# Autodesk Inventor assembly: Main_assembly
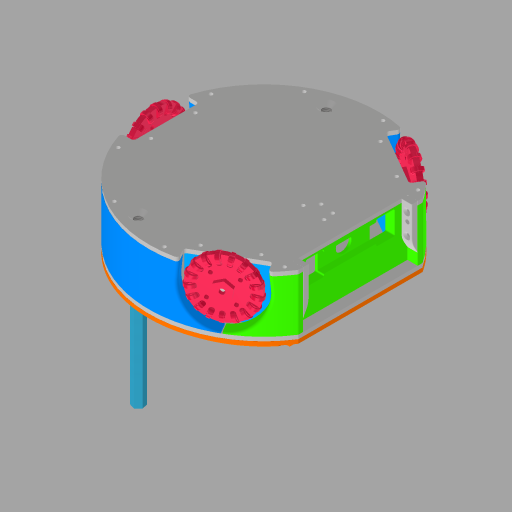
[picture p0: Inventor's stored thumbnail of the model, 512x512]
Saved by Autodesk Inventor 2024.2 (Build 282272000, 272)
## iProperties
Created: 2024-03-14
Part Number: Main_assembly
Document SubType Name: Assembly
Designer: Fedor Orlov
Author: Fedor Orlov
## Documents named in this file (18)
- C:\Users\Fedor Orlov\OneDrive\Robocup SSL\3D model\Main_assembly.iam
- C:\Users\Fedor Orlov\OneDrive\Robocup SSL\3D model\Level_1.ipt
- C:\Users\Fedor Orlov\OneDrive\Robocup SSL\3D model\Motor_mounting.ipt
- C:\Users\Fedor Orlov\OneDrive\Robocup SSL\3D model\Motor_mounting_left.ipt
- C:\Users\Fedor Orlov\OneDrive\Robocup SSL\3D model\Stand_M3_40mm.ipt
- C:\Users\Fedor Orlov\OneDrive\Robocup SSL\3D model\Stand_M6_40mm.ipt
- C:\Users\Fedor Orlov\OneDrive\Robocup SSL\3D model\Lower_protection_left.ipt
- C:\Users\Fedor Orlov\OneDrive\Robocup SSL\3D model\25d-metal-gearmotor-20.4.ipt
- C:\Users\Fedor Orlov\OneDrive\Robocup SSL\3D model\Lower_protection_right.ipt
- C:\Users\Fedor Orlov\OneDrive\Robocup SSL\3D model\gtf robots 50mm.ipt
- C:\Users\Fedor Orlov\OneDrive\Robocup SSL\3D model\Lower_protection_front.ipt
- C:\Users\Fedor Orlov\OneDrive\Robocup SSL\3D model\Level_2.ipt
- C:\Users\Fedor Orlov\OneDrive\Robocup SSL\3D model\LED_mounting_right.ipt
- C:\Users\Fedor Orlov\OneDrive\Robocup SSL\3D model\LED_mounting_left.ipt
- C:\Users\Fedor Orlov\OneDrive\Robocup SSL\3D model\Lid_lock.ipt
- C:\Users\Fedor Orlov\OneDrive\Robocup SSL\3D model\Capacitor_board_assembly.iam
- C:\Users\Fedor Orlov\OneDrive\Robocup SSL\3D model\Stand_M4_40mm.ipt
- C:\Users\Fedor Orlov\OneDrive\Robocup SSL\3D model\Stand_M6_80mm.ipt
## Components (31 placed, 17 different names)
1. Level_1:1 — Совмещение:1, Совмещение:2, Совмещение:3, Заподлицо:1, Заподлицо:2, Заподлицо:3, Совмещение:4, Совмещение:5, Совмещение:6, Совмещение:7, Совмещение:8, Совмещение:9, Совмещение:10, Совмещение:11, Совмещение:12, Совмещение:13, Совмещение:14, Совмещение:15, Совмещение:16, Совмещение:17, Совмещение:18, Совмещение:19, Совмещение:20, Совмещение:21, Совмещение:22, Совмещение:23, Совмещение:24, Совмещение:25, Совмещение:26, Совмещение:27, Совмещение:28, Заподлицо:4, Совмещение:29, Совмещение:30, Совмещение:31, Совмещение:41, Совмещение:42, Совмещение:43, Совмещение:50, Заподлицо:5, Совмещение:51, Совмещение:53
2. Motor_mounting:1 — Совмещение:1, Заподлицо:3, Совмещение:4, Совмещение:32, Совмещение:37, Совмещение:38, Совмещение:49
3. Motor_mounting:2 — Совмещение:2, Заподлицо:2, Совмещение:5, Совмещение:33, Совмещение:36, Совмещение:39, Совмещение:48
4. Motor_mounting_left:1 — Совмещение:3, Заподлицо:1, Совмещение:6, Совмещение:34, Совмещение:35, Совмещение:40, Совмещение:47
5. Stand_M3_40mm:1 — Совмещение:9, Совмещение:10, Угол:8, Совмещение:54
6. Stand_M3_40mm:2 — Совмещение:7, Совмещение:8, Угол:7
7. Stand_M3_40mm:3 — Совмещение:21, Совмещение:22, Угол:6
8. Stand_M3_40mm:4 — Совмещение:19, Совмещение:20, Угол:5
9. Stand_M3_40mm:5 — Совмещение:17, Совмещение:18, Угол:4
10. Stand_M3_40mm:6 — Совмещение:15, Совмещение:16, Угол:3
11. Stand_M3_40mm:7 — Совмещение:13, Совмещение:14, Угол:2
12. Stand_M3_40mm:8 — Совмещение:11, Совмещение:12, Угол:1
13. Stand_M6_40mm:1 — Совмещение:23, Совмещение:24
14. Stand_M6_40mm:2 — Совмещение:25, Совмещение:26
15. Lower_protection_left:1 — Совмещение:29, Совмещение:30, Совмещение:31, Угол:1, Угол:2, Угол:3, Совмещение:62
16. 25d-metal-gearmotor-20.4:1 — Совмещение:32, Совмещение:37, Совмещение:38, Совмещение:45
17. 25d-metal-gearmotor-20.4:2 — Совмещение:34, Совмещение:35, Совмещение:40, Совмещение:46
18. 25d-metal-gearmotor-20.4:3 — Совмещение:33, Совмещение:36, Совмещение:39, Совмещение:44
19. Lower_protection_right:1 — Совмещение:41, Совмещение:42, Совмещение:43, Угол:4, Угол:5, Угол:6
20. gtf robots 50mm:1 — Совмещение:44, Совмещение:48
21. gtf robots 50mm:2 — Совмещение:46, Совмещение:47
22. gtf robots 50mm:3 — Совмещение:45, Совмещение:49
23. Lower_protection_front:1 — Совмещение:50, Заподлицо:5, Совмещение:51, Угол:7, Угол:8, Совмещение:52, Совмещение:55, Совмещение:56, Совмещение:57, Совмещение:58, Совмещение:59, Совмещение:60
24. Level_2:1 — Совмещение:52, Совмещение:53, Совмещение:54, Совмещение:61, Заподлицо:6, Совмещение:63, Совмещение:64, Совмещение:65, Совмещение:66, Совмещение:67, Совмещение:68, Совмещение:69, Совмещение:70, Совмещение:71
25. LED_mounting_right:1 — Совмещение:55, Совмещение:56, Совмещение:57
26. LED_mounting_left:1 — Совмещение:58, Совмещение:59, Совмещение:60
27. Lid_lock:1 — Совмещение:61, Совмещение:62, Заподлицо:6
28. Capacitor_board_assembly:1 [sub-assembly] — Совмещение:63, Совмещение:64, Совмещение:65
29. Stand_M4_40mm:1 — Совмещение:66, Совмещение:67
30. Stand_M6_80mm:1 — Совмещение:68, Совмещение:71
31. Stand_M6_80mm:2 — Совмещение:69, Совмещение:70
## Relationships (85: Mate 71, Angle 8, Flush 6)
- Совмещение:1 [Mate]: Level_1:1 ↔ Motor_mounting:1
- Совмещение:2 [Mate]: Level_1:1 ↔ Motor_mounting:2
- Совмещение:3 [Mate]: Level_1:1 ↔ Motor_mounting_left:1
- Заподлицо:1 [Flush]: Level_1:1 ↔ Motor_mounting_left:1
- Заподлицо:2 [Flush]: Level_1:1 ↔ Motor_mounting:2
- Заподлицо:3 [Flush]: Level_1:1 ↔ Motor_mounting:1
- Совмещение:4 [Mate]: Level_1:1 ↔ Motor_mounting:1
- Совмещение:5 [Mate]: Level_1:1 ↔ Motor_mounting:2
- Совмещение:6 [Mate]: Level_1:1 ↔ Motor_mounting_left:1
- Совмещение:7 [Mate]: Level_1:1 ↔ Stand_M3_40mm:2
- Совмещение:8 [Mate]: Level_1:1 ↔ Stand_M3_40mm:2
- Совмещение:9 [Mate]: Level_1:1 ↔ Stand_M3_40mm:1
- Совмещение:10 [Mate]: Level_1:1 ↔ Stand_M3_40mm:1
- Совмещение:11 [Mate]: Level_1:1 ↔ Stand_M3_40mm:8
- Совмещение:12 [Mate]: Level_1:1 ↔ Stand_M3_40mm:8
- Совмещение:13 [Mate]: Level_1:1 ↔ Stand_M3_40mm:7
- Совмещение:14 [Mate]: Level_1:1 ↔ Stand_M3_40mm:7
- Совмещение:15 [Mate]: Level_1:1 ↔ Stand_M3_40mm:6
- Совмещение:16 [Mate]: Level_1:1 ↔ Stand_M3_40mm:6
- Совмещение:17 [Mate]: Level_1:1 ↔ Stand_M3_40mm:5
- Совмещение:18 [Mate]: Level_1:1 ↔ Stand_M3_40mm:5
- Совмещение:19 [Mate]: Level_1:1 ↔ Stand_M3_40mm:4
- Совмещение:20 [Mate]: Level_1:1 ↔ Stand_M3_40mm:4
- Совмещение:21 [Mate]: Level_1:1 ↔ Stand_M3_40mm:3
- Совмещение:22 [Mate]: Level_1:1 ↔ Stand_M3_40mm:3
- Совмещение:23 [Mate]: Level_1:1 ↔ Stand_M6_40mm:1
- Совмещение:24 [Mate]: Level_1:1 ↔ Stand_M6_40mm:1
- Совмещение:25 [Mate]: Level_1:1 ↔ Stand_M6_40mm:2
- Совмещение:26 [Mate]: Level_1:1 ↔ Stand_M6_40mm:2
- Совмещение:27 [Mate]: Level_1:1
- Совмещение:28 [Mate]: Level_1:1
- Заподлицо:4 [Flush]: Level_1:1
- Совмещение:29 [Mate]: Level_1:1 ↔ Lower_protection_left:1
- Совмещение:30 [Mate]: Level_1:1 ↔ Lower_protection_left:1
- Совмещение:31 [Mate]: Level_1:1 ↔ Lower_protection_left:1
- Угол:1 [Angle] (0 deg): Stand_M3_40mm:8 ↔ Lower_protection_left:1
- Угол:2 [Angle] (0 deg): Stand_M3_40mm:7 ↔ Lower_protection_left:1
- Угол:3 [Angle] (0 deg): Stand_M3_40mm:6 ↔ Lower_protection_left:1
- Совмещение:32 [Mate]: Motor_mounting:1 ↔ 25d-metal-gearmotor-20.4:1
- Совмещение:33 [Mate]: Motor_mounting:2 ↔ 25d-metal-gearmotor-20.4:3
- Совмещение:34 [Mate]: Motor_mounting_left:1 ↔ 25d-metal-gearmotor-20.4:2
- Совмещение:35 [Mate]: Motor_mounting_left:1 ↔ 25d-metal-gearmotor-20.4:2
- Совмещение:36 [Mate]: Motor_mounting:2 ↔ 25d-metal-gearmotor-20.4:3
- Совмещение:37 [Mate]: Motor_mounting:1 ↔ 25d-metal-gearmotor-20.4:1
- Совмещение:38 [Mate]: Motor_mounting:1 ↔ 25d-metal-gearmotor-20.4:1
- Совмещение:39 [Mate]: Motor_mounting:2 ↔ 25d-metal-gearmotor-20.4:3
- Совмещение:40 [Mate]: Motor_mounting_left:1 ↔ 25d-metal-gearmotor-20.4:2
- Совмещение:41 [Mate]: Level_1:1 ↔ Lower_protection_right:1
- Совмещение:42 [Mate]: Level_1:1 ↔ Lower_protection_right:1
- Совмещение:43 [Mate]: Level_1:1 ↔ Lower_protection_right:1
- Совмещение:44 [Mate]: 25d-metal-gearmotor-20.4:3 ↔ gtf robots 50mm:1
- Совмещение:45 [Mate]: 25d-metal-gearmotor-20.4:1 ↔ gtf robots 50mm:3
- Совмещение:46 [Mate]: 25d-metal-gearmotor-20.4:2 ↔ gtf robots 50mm:2
- Совмещение:47 [Mate]: Motor_mounting_left:1 ↔ gtf robots 50mm:2
- Совмещение:48 [Mate]: Motor_mounting:2 ↔ gtf robots 50mm:1
- Совмещение:49 [Mate]: Motor_mounting:1 ↔ gtf robots 50mm:3
- Совмещение:50 [Mate]: Level_1:1 ↔ Lower_protection_front:1
- Заподлицо:5 [Flush]: Level_1:1 ↔ Lower_protection_front:1
- Совмещение:51 [Mate]: Level_1:1 ↔ Lower_protection_front:1
- Угол:4 [Angle] (0 deg): Stand_M3_40mm:5 ↔ Lower_protection_right:1
- Угол:5 [Angle] (0 deg): Stand_M3_40mm:4 ↔ Lower_protection_right:1
- Угол:6 [Angle] (0 deg): Stand_M3_40mm:3 ↔ Lower_protection_right:1
- Угол:7 [Angle] (0 deg): Stand_M3_40mm:2 ↔ Lower_protection_front:1
- Угол:8 [Angle] (0 deg): Stand_M3_40mm:1 ↔ Lower_protection_front:1
- Совмещение:52 [Mate]: Lower_protection_front:1 ↔ Level_2:1
- Совмещение:53 [Mate]: Level_1:1 ↔ Level_2:1
- Совмещение:54 [Mate]: Stand_M3_40mm:1 ↔ Level_2:1
- Совмещение:55 [Mate]: Lower_protection_front:1 ↔ LED_mounting_right:1
- Совмещение:56 [Mate]: Lower_protection_front:1 ↔ LED_mounting_right:1
- Совмещение:57 [Mate]: Lower_protection_front:1 ↔ LED_mounting_right:1
- Совмещение:58 [Mate]: Lower_protection_front:1 ↔ LED_mounting_left:1
- Совмещение:59 [Mate]: Lower_protection_front:1 ↔ LED_mounting_left:1
- Совмещение:60 [Mate]: Lower_protection_front:1 ↔ LED_mounting_left:1
- Совмещение:61 [Mate]: Level_2:1 ↔ Lid_lock:1
- Совмещение:62 [Mate]: Lower_protection_left:1 ↔ Lid_lock:1
- Заподлицо:6 [Flush]: Level_2:1 ↔ Lid_lock:1
- Совмещение:63 [Mate]: Level_2:1 ↔ Capacitor_board_assembly:1
- Совмещение:64 [Mate]: Level_2:1 ↔ Capacitor_board_assembly:1
- Совмещение:65 [Mate]: Level_2:1 ↔ Capacitor_board_assembly:1
- Совмещение:66 [Mate]: Level_2:1 ↔ Stand_M4_40mm:1
- Совмещение:67 [Mate]: Level_2:1 ↔ Stand_M4_40mm:1
- Совмещение:68 [Mate]: Level_2:1 ↔ Stand_M6_80mm:1
- Совмещение:69 [Mate]: Level_2:1 ↔ Stand_M6_80mm:2
- Совмещение:70 [Mate]: Level_2:1 ↔ Stand_M6_80mm:2
- Совмещение:71 [Mate]: Level_2:1 ↔ Stand_M6_80mm:1
